# Autodesk Inventor assembly: front_motor_gear
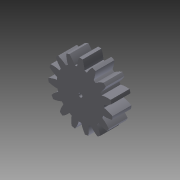
[picture p0: Inventor's stored thumbnail of the model, 180x180]
Saved by Autodesk Inventor 2015 (Build 190159000, 159)
## iProperties
Created: 2015-06-18
Part Number: front_motor_gear
Document SubType Name: Assembly
Designer: Abhishyant
Author: Abhishyant
## Documents named in this file (3)
- D:\Projects\Personal\BroBot\3D Model\front_motor_gear.iam
- D:\Projects\Personal\BroBot\3D Model\motor_gear_hole_maker.ipt
- D:\Projects\Personal\BroBot\3D Model\front_motor_gear\Design Accelerator\Spur Gears1.iam
## Components (2 placed, 2 different names)
1. motor_gear_hole_maker:1 — Mate:1
2. Spur Gears:1 [sub-assembly] — Mate:1
## Relationships (1: Mate 1)
- Mate:1: motor_gear_hole_maker:1 ↔ Spur Gears:1
